# Autodesk Inventor assembly: main assembly
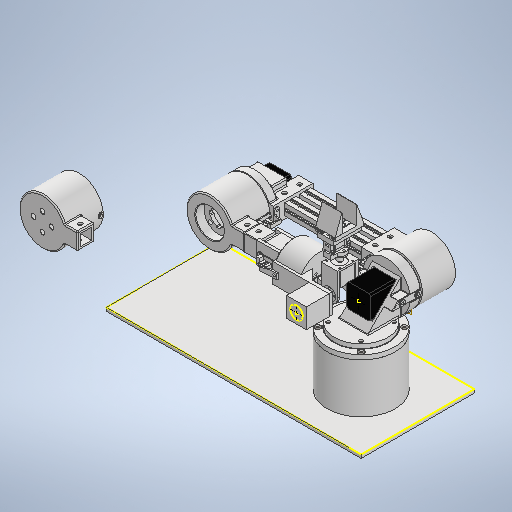
[picture p0: Inventor's stored thumbnail of the model, 512x512]
Saved by Autodesk Inventor 2025 (Build 290162000, 162)
## iProperties
Created: 2025-07-04
Part Number: main assembly
Document SubType Name: Assembly
Designer: gavin
Author: gavin
## Documents named in this file (35)
- D:\Inventor\robot armT 2\main assembly.iam
- D:\Inventor\robot armT 2\stepper 42x48 - 27.ipt
- D:\Inventor\robot armT 2\28stepper27.ipt
- D:\Inventor\robot armT 2\CSN 02 4630 - 6009.ipt
- D:\Inventor\robot armT 2\CNS 2862 B2116 - 6007 - 35 x 62 x 14.ipt
- D:\Inventor\robot armT 2\base plate.ipt
- D:\Inventor\robot armT 2\stepper 42x60 -50 .ipt
- D:\Inventor\robot armT 2\j2 42 motor mount.ipt
- D:\Inventor\robot armT 2\j2 arm part.ipt
- D:\Inventor\robot armT 2\j1 assmble.iam
- D:\Inventor\robot armT 2\optic endstop module.ipt
- D:\Inventor\robot armT 2\j2j3 alumi ext.ipt
- D:\Inventor\robot armT 2\j3 motor mount.ipt
- D:\Inventor\robot armT 2\j3 moving part.ipt
- D:\Inventor\robot armT 2\j3j4 alumi ext.ipt
- D:\Inventor\robot armT 2\j2 endstop blocker.ipt
- D:\Inventor\robot armT 2\j3 endstop blocker.ipt
- D:\Inventor\robot armT 2\6mm axle hub.ipt
- D:\Inventor\robot armT 2\j4 motor mount.ipt
- D:\Inventor\robot armT 2\j4 motor mount cover.ipt
- D:\Inventor\robot armT 2\j4 moving part.ipt
- D:\Inventor\robot armT 2\nema 11x25.ipt
- D:\Inventor\robot armT 2\5mm axle hub.ipt
- D:\Inventor\robot armT 2\bearing 22-M6.ipt
- D:\Inventor\robot armT 2\j6 motor mount v2.ipt
- D:\Inventor\robot armT 2\j4 endstop blocker.ipt
- D:\Inventor\Tugofwarv2\z11-8x15 axle mount.ipt
- D:\Inventor\Tugofwarv2\j2 mount plate.ipt
- D:\Inventor\robot armT 2\sg90 long claw.iam
- D:\Inventor\robot armT 2\j3 moving part 2 option.ipt
- D:\Inventor\robot armT 2\35x40 stepper.ipt
- D:\Inventor\robot armT 2\j3 moving part option3.ipt
- D:\Inventor\robot armT 2\z21 8x18.ipt
- D:\Inventor\robot armT 2\18mm hub.ipt
- D:\Inventor\robot armT 2\j2 moving part option2.ipt
## Components (43 placed, 34 different names)
1. base plate:1 — 齊平:5
2. j1 assmble:1 [sub-assembly]
3. stepper 42x48 - 27:2 — 貼合:45, 貼合:46, 貼合:47, 貼合:94, 貼合:110, 齊平:18
4. CSN 02 4630 - 6009:1 — 貼合:48, 貼合:49, 貼合:50, 貼合:51, 貼合:111, 齊平:19
5. CSN 02 4630 - 6009:2 — 貼合:16, 貼合:29, 貼合:30, 貼合:31, 貼合:114
6. CNS 2862 B2116 - 6007 - 35 x 62 x 14:1 — 貼合:63, 貼合:64, 貼合:75, 齊平:17
7. stepper 42x60 -50 :1 — 貼合:16, 貼合:27, 貼合:28, 貼合:92, 貼合:113, 齊平:20
8. j2 42 motor mount:1 — 貼合:27, 貼合:28, 貼合:29, 貼合:33, 貼合:34, 貼合:35, 貼合:93
9. j2 arm part:1 — 貼合:30, 貼合:31, 貼合:36, 貼合:37, 貼合:38, 貼合:39, 貼合:40, 貼合:41, 齊平:9
10. optic endstop module:1 — 貼合:33, 貼合:34, 貼合:35, 齊平:10
11. j2j3 alumi ext:1 — 貼合:36, 貼合:37, 貼合:38, 貼合:42, 貼合:43, 貼合:44, 齊平:13
12. j2j3 alumi ext:2 — 貼合:39, 貼合:40, 貼合:41, 貼合:116
13. j3 motor mount:1 — 貼合:42, 貼合:43, 貼合:44, 貼合:45, 貼合:46, 貼合:47, 貼合:48, 貼合:49, 齊平:11, 齊平:12, 貼合:59, 貼合:95
14. j3 moving part:1 — 貼合:50, 貼合:51, 貼合:52, 貼合:53, 貼合:54, 貼合:55, 貼合:56, 貼合:57
15. j3j4 alumi ext:1 — 貼合:52, 貼合:53, 貼合:54, 齊平:13, 貼合:68, 貼合:69, 貼合:70
16. optic endstop module:2 — 貼合:55, 貼合:56, 貼合:57, 貼合:58
17. j2 endstop blocker:1 — 齊平:9, 齊平:10
18. j3 endstop blocker:1 — 齊平:11, 齊平:12, 貼合:58, 貼合:59
19. 6mm axle hub:1 — 旋轉:13, 貼合:106
20. j4 motor mount:1 — 齊平:14, 齊平:15, 貼合:60, 貼合:61, 貼合:62, 貼合:63, 貼合:65, 貼合:68, 貼合:69, 貼合:70, 貼合:71, 貼合:72, 貼合:73
21. j4 motor mount cover:1 — 齊平:14, 齊平:15, 貼合:62, 貼合:64, 貼合:65
22. 28stepper27:1 — 貼合:60, 貼合:61, 旋轉:13
23. optic endstop module:3 — 貼合:71, 貼合:72, 貼合:73
24. j4 moving part:1 — 貼合:74, 貼合:75, 齊平:17, 貼合:76, 貼合:86, 貼合:87, 貼合:104, 貼合:105, 貼合:106, 貼合:107, 貼合:108, 貼合:109
25. nema 11x25:1 — 貼合:88, 貼合:89, 貼合:102, 貼合:103
26. optic endstop module:4 — 貼合:74, 貼合:76, 貼合:107
27. 5mm axle hub:1 — 剛性:1, 旋轉:12
28. bearing 22-M6:1 — 貼合:86, 貼合:87
29. j6 motor mount v2:1 — 貼合:88, 貼合:89, 旋轉:12
30. j4 endstop blocker:1 — 貼合:108, 貼合:109
31. z11-8x15 axle mount:1 — 貼合:92, 貼合:93, 貼合:96, 貼合:97, 貼合:98
32. z11-8x15 axle mount:2 — 貼合:94, 貼合:95
33. j2 mount plate:1 — 貼合:96, 貼合:97, 貼合:98
34. sg90 long claw:1 [sub-assembly] — 貼合:99, 貼合:100, 貼合:101, 貼合:103
35. 5mm axle hub:2 — 貼合:99, 貼合:100, 貼合:101, 貼合:102
36. j3 moving part 2 option:1
37. 35x40 stepper:1 — 貼合:104, 貼合:105, 剛性:1
38. j3 moving part option3:1 — 貼合:111, 齊平:19, 貼合:112
39. z21 8x18:1 — 剛性:2, 貼合:110, 齊平:18
40. 18mm hub:1 — 剛性:2, 貼合:112
41. j2 moving part option2:1 — 貼合:114, 貼合:115, 貼合:116
42. z21 8x18:2 — 貼合:113, 齊平:20
43. 18mm hub:2 — 貼合:115
## Relationships (109: Mate 84, Flush 14, RevoluteJoint 8, WeldJoint 3)
- [Mate]: j1 assmble:1
- [Flush]: base plate:1 ↔ j1 assmble:1
- [Mate]: base plate:1 ↔ j1 assmble:1
- 齊平:5 [Flush]: base plate:1
- 貼合:16 [Mate]: CSN 02 4630 - 6009:2 ↔ stepper 42x60 -50 :1
- [Mate] (20 mm): j1 assmble:1 ↔ stepper 42x60 -50 :1
- [Mate]: j1 assmble:1 ↔ j2 42 motor mount:1
- [Mate]: base plate:1 ↔ j1 assmble:1
- [Mate]: j1 assmble:1 ↔ j2 42 motor mount:1
- [Mate]: j1 assmble:1 ↔ j2 42 motor mount:1
- 貼合:27 [Mate]: stepper 42x60 -50 :1 ↔ j2 42 motor mount:1
- 貼合:28 [Mate]: stepper 42x60 -50 :1 ↔ j2 42 motor mount:1
- 貼合:29 [Mate]: CSN 02 4630 - 6009:2 ↔ j2 42 motor mount:1
- 貼合:30 [Mate]: CSN 02 4630 - 6009:2 ↔ j2 arm part:1
- [Flush] (-56.075 mm): j1 assmble:1 ↔ j2 arm part:1
- 貼合:31 [Mate]: CSN 02 4630 - 6009:2 ↔ j2 arm part:1
- [RevoluteJoint]: base plate:1 ↔ j1 assmble:1
- [RevoluteJoint]: base plate:1 ↔ j1 assmble:1
- [RevoluteJoint]: base plate:1 ↔ j1 assmble:1
- [RevoluteJoint]: base plate:1 ↔ j1 assmble:1
- [RevoluteJoint]: base plate:1 ↔ j1 assmble:1
- [RevoluteJoint]: base plate:1 ↔ j1 assmble:1
- 貼合:33 [Mate]: j2 42 motor mount:1 ↔ optic endstop module:1
- 貼合:34 [Mate]: j2 42 motor mount:1 ↔ optic endstop module:1
- 貼合:35 [Mate]: j2 42 motor mount:1 ↔ optic endstop module:1
- 貼合:36 [Mate]: j2 arm part:1 ↔ j2j3 alumi ext:1
- 貼合:37 [Mate] (0.075 mm): j2 arm part:1 ↔ j2j3 alumi ext:1
- 貼合:38 [Mate] (0.075 mm): j2 arm part:1 ↔ j2j3 alumi ext:1
- 貼合:39 [Mate]: j2 arm part:1 ↔ j2j3 alumi ext:2
- 貼合:40 [Mate] (0.075 mm): j2 arm part:1 ↔ j2j3 alumi ext:2
- 貼合:41 [Mate] (0.075 mm): j2 arm part:1 ↔ j2j3 alumi ext:2
- 貼合:42 [Mate]: j2j3 alumi ext:1 ↔ j3 motor mount:1
- 貼合:43 [Mate] (0.075 mm): j2j3 alumi ext:1 ↔ j3 motor mount:1
- 貼合:44 [Mate] (0.075 mm): j2j3 alumi ext:1 ↔ j3 motor mount:1
- 貼合:45 [Mate]: stepper 42x48 - 27:2 ↔ j3 motor mount:1
- 貼合:46 [Mate] (0.075 mm): stepper 42x48 - 27:2 ↔ j3 motor mount:1
- 貼合:47 [Mate]: stepper 42x48 - 27:2 ↔ j3 motor mount:1
- 貼合:48 [Mate]: CSN 02 4630 - 6009:1 ↔ j3 motor mount:1
- 貼合:49 [Mate]: CSN 02 4630 - 6009:1 ↔ j3 motor mount:1
- 貼合:50 [Mate]: CSN 02 4630 - 6009:1 ↔ j3 moving part:1
- 貼合:51 [Mate]: CSN 02 4630 - 6009:1 ↔ j3 moving part:1
- 貼合:52 [Mate] (0.075 mm): j3 moving part:1 ↔ j3j4 alumi ext:1
- 貼合:53 [Mate]: j3 moving part:1 ↔ j3j4 alumi ext:1
- 貼合:54 [Mate] (0.075 mm): j3 moving part:1 ↔ j3j4 alumi ext:1
- 貼合:55 [Mate]: j3 moving part:1 ↔ optic endstop module:2
- 貼合:56 [Mate]: j3 moving part:1 ↔ optic endstop module:2
- 貼合:57 [Mate]: j3 moving part:1 ↔ optic endstop module:2
- 齊平:9 [Flush]: j2 arm part:1 ↔ j2 endstop blocker:1
- 齊平:10 [Flush]: optic endstop module:1 ↔ j2 endstop blocker:1
- 齊平:11 [Flush]: j3 motor mount:1 ↔ j3 endstop blocker:1
- 齊平:12 [Flush]: j3 motor mount:1 ↔ j3 endstop blocker:1
- 貼合:58 [Mate]: optic endstop module:2 ↔ j3 endstop blocker:1
- 齊平:13 [Flush]: j2j3 alumi ext:1 ↔ j3j4 alumi ext:1
- 齊平:14 [Flush]: j4 motor mount:1 ↔ j4 motor mount cover:1
- 齊平:15 [Flush]: j4 motor mount:1 ↔ j4 motor mount cover:1
- 貼合:59 [Mate]: j3 motor mount:1 ↔ j3 endstop blocker:1
- 貼合:60 [Mate]: j4 motor mount:1 ↔ 28stepper27:1
- 貼合:61 [Mate]: j4 motor mount:1 ↔ 28stepper27:1
- 貼合:62 [Mate]: j4 motor mount:1 ↔ j4 motor mount cover:1
- 貼合:63 [Mate]: CNS 2862 B2116 - 6007 - 35 x 62 x 14:1 ↔ j4 motor mount:1
- 貼合:64 [Mate]: CNS 2862 B2116 - 6007 - 35 x 62 x 14:1 ↔ j4 motor mount cover:1
- 貼合:65 [Mate]: j4 motor mount:1 ↔ j4 motor mount cover:1
- 貼合:68 [Mate]: j3j4 alumi ext:1 ↔ j4 motor mount:1
- 貼合:69 [Mate] (0.075 mm): j3j4 alumi ext:1 ↔ j4 motor mount:1
- 貼合:70 [Mate] (0.075 mm): j3j4 alumi ext:1 ↔ j4 motor mount:1
- 貼合:71 [Mate]: j4 motor mount:1 ↔ optic endstop module:3
- 貼合:72 [Mate]: j4 motor mount:1 ↔ optic endstop module:3
- 貼合:73 [Mate]: j4 motor mount:1 ↔ optic endstop module:3
- 貼合:74 [Mate]: j4 moving part:1 ↔ optic endstop module:4
- 貼合:75 [Mate]: CNS 2862 B2116 - 6007 - 35 x 62 x 14:1 ↔ j4 moving part:1
- 齊平:17 [Flush]: CNS 2862 B2116 - 6007 - 35 x 62 x 14:1 ↔ j4 moving part:1
- 貼合:76 [Mate]: j4 moving part:1 ↔ optic endstop module:4
- 貼合:86 [Mate]: j4 moving part:1 ↔ bearing 22-M6:1
- 貼合:87 [Mate]: j4 moving part:1 ↔ bearing 22-M6:1
- 貼合:88 [Mate]: nema 11x25:1 ↔ j6 motor mount v2:1
- 貼合:89 [Mate]: nema 11x25:1 ↔ j6 motor mount v2:1
- 貼合:92 [Mate]: stepper 42x60 -50 :1 ↔ z11-8x15 axle mount:1
- 貼合:93 [Mate]: j2 42 motor mount:1 ↔ z11-8x15 axle mount:1
- 貼合:94 [Mate]: stepper 42x48 - 27:2 ↔ z11-8x15 axle mount:2
- 貼合:95 [Mate]: j3 motor mount:1 ↔ z11-8x15 axle mount:2
- 貼合:96 [Mate]: z11-8x15 axle mount:1 ↔ j2 mount plate:1
- 貼合:97 [Mate]: z11-8x15 axle mount:1 ↔ j2 mount plate:1
- 貼合:98 [Mate]: z11-8x15 axle mount:1 ↔ j2 mount plate:1
- 貼合:99 [Mate]: sg90 long claw:1 ↔ 5mm axle hub:2
- 貼合:100 [Mate]: sg90 long claw:1 ↔ 5mm axle hub:2
- 貼合:101 [Mate]: sg90 long claw:1 ↔ 5mm axle hub:2
- 貼合:102 [Mate]: nema 11x25:1 ↔ 5mm axle hub:2
- 貼合:103 [Mate]: nema 11x25:1 ↔ sg90 long claw:1
- 貼合:104 [Mate]: j4 moving part:1 ↔ 35x40 stepper:1
- 貼合:105 [Mate]: j4 moving part:1 ↔ 35x40 stepper:1
- 剛性:1 [WeldJoint]: 5mm axle hub:1 ↔ 35x40 stepper:1
- 旋轉:12 [RevoluteJoint]: 5mm axle hub:1 ↔ j6 motor mount v2:1
- 旋轉:13 [RevoluteJoint]: 6mm axle hub:1 ↔ 28stepper27:1
- 貼合:106 [Mate]: 6mm axle hub:1 ↔ j4 moving part:1
- 貼合:107 [Mate]: j4 moving part:1 ↔ optic endstop module:4
- 貼合:108 [Mate]: j4 moving part:1 ↔ j4 endstop blocker:1
- 貼合:109 [Mate]: j4 moving part:1 ↔ j4 endstop blocker:1
- 剛性:2 [WeldJoint] (-3.71 mm): z21 8x18:1 ↔ 18mm hub:1
- 貼合:110 [Mate]: stepper 42x48 - 27:2 ↔ z21 8x18:1
- 齊平:18 [Flush]: stepper 42x48 - 27:2 ↔ z21 8x18:1
- 貼合:111 [Mate]: CSN 02 4630 - 6009:1 ↔ j3 moving part option3:1
- 齊平:19 [Flush]: CSN 02 4630 - 6009:1 ↔ j3 moving part option3:1
- 貼合:112 [Mate]: j3 moving part option3:1 ↔ 18mm hub:1
- [WeldJoint] (-3.71 mm): z21 8x18:2 ↔ 18mm hub:2
- 貼合:113 [Mate]: stepper 42x60 -50 :1 ↔ z21 8x18:2
- 齊平:20 [Flush]: stepper 42x60 -50 :1 ↔ z21 8x18:2
- 貼合:114 [Mate]: CSN 02 4630 - 6009:2 ↔ j2 moving part option2:1
- 貼合:115 [Mate]: j2 moving part option2:1 ↔ 18mm hub:2
- 貼合:116 [Mate] (0.075 mm): j2j3 alumi ext:2 ↔ j2 moving part option2:1
## Named parameters: d225_d219 = -3.71 mm
